# Autodesk Inventor assembly: UVTRONassembly
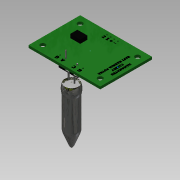
[picture p0: Inventor's stored thumbnail of the model, 180x180]
Saved by Autodesk Inventor 2015 SP1 (Build 190203100, 203)
## iProperties
Created: 2015-01-27
Part Number: UVTRONassembly
Document SubType Name: Assembly
Designer: Rafi Kurnia Putra
Author: Rafi Kurnia Putra
## Documents named in this file (3)
- D:\Dropbox\krpai berkaki trui 2015\ROBUSTA\MEKANIK\ROBUSTA\Assembly UVTRON.iam
- D:\Dropbox\krpai berkaki trui 2015\ROBUSTA\MEKANIK\ROBUSTA\UVTRON.ipt
- D:\Dropbox\krpai berkaki trui 2015\ROBUSTA\MEKANIK\ROBUSTA\Buble UVTRON.ipt
## Components (2 placed, 2 different names)
1. UVTRON:1 — Mate:1, Mate:2, Mate:3, Mate:4, Flush:1, Flush:2
2. Buble UVTRON:1 — Mate:1, Mate:2, Flush:2
## Relationships (6: Mate 4, Flush 2)
- Mate:1: UVTRON:1 ↔ Buble UVTRON:1
- Mate:2: UVTRON:1 ↔ Buble UVTRON:1
- Mate:3: UVTRON:1
- Mate:4: UVTRON:1
- Flush:1: UVTRON:1
- Flush:2 (-1 mm): UVTRON:1 ↔ Buble UVTRON:1
